# Autodesk Inventor assembly: Model-3
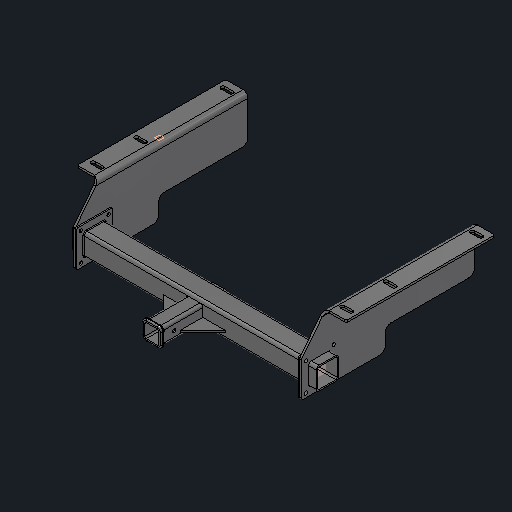
[picture p0: Inventor's stored thumbnail of the model, 512x512]
Saved by Autodesk Inventor 2025.1 (Build 291241000, 241)
## iProperties
Created: 2026-02-13
Part Number: Model-3
Document SubType Name: Assembly
Designer: Desktop -24
Mass: 20583.6 g
Surface Area: 8150.6 cm^2
Volume: 2573.11 cm^3
Density: 7.99949 g/cm^3
encoded128: ÌStandard (in)rÎ
Family: ASSEMBLY
Author: Desktop -24
## Documents named in this file (6)
- F:\OneDrive - nLeague Technologies Private Limited\Desktop\Sharath Chandra\Rear Hitch\Model-3\Model-3.iam
- F:\OneDrive - nLeague Technologies Private Limited\Desktop\Sharath Chandra\Rear Hitch\Model-3\Model-3_Base Tube-1.ipt
- F:\OneDrive - nLeague Technologies Private Limited\Desktop\Sharath Chandra\Rear Hitch\Model-3\Model-3_Sheet-LH.ipt
- F:\OneDrive - nLeague Technologies Private Limited\Desktop\Sharath Chandra\Rear Hitch\Model-3\Model-3_Sheet-RH.ipt
- F:\OneDrive - nLeague Technologies Private Limited\Desktop\Sharath Chandra\Rear Hitch\Model-3\Model-3_Base Tube-2.ipt
- F:\OneDrive - nLeague Technologies Private Limited\Desktop\Sharath Chandra\Rear Hitch\Model-3\Model-3_Sheet Stifferner.ipt
## Components (6 placed, 5 different names)
1. Model-3_Sheet-LH:1 — Mate:14, Flush:13, Flush:14
2. Model-3_Base Tube-1:1 — Mate:4, Mate:5, Flush:2, Mate:8, Mate:10, Mate:13, Flush:11, Flush:12, Mate:14, Flush:13, Flush:14
3. Model-3_Base Tube-2:1 — Mate:4, Mate:5, Flush:2, Mate:9, Mate:11, Flush:8
4. Model-3_Sheet-RH:1 — Mate:13, Flush:11, Flush:12
5. Model-3_Sheet Stifferner:1 — Mate:8, Mate:9, Flush:7
6. Model-3_Sheet Stifferner:2 — Mate:10, Mate:11, Flush:7, Flush:8
## Relationships (15: Mate 8, Flush 7)
- Mate:4: Model-3_Base Tube-1:1 ↔ Model-3_Base Tube-2:1
- Mate:5: Model-3_Base Tube-1:1 ↔ Model-3_Base Tube-2:1
- Flush:2 (9.525 mm): Model-3_Base Tube-1:1 ↔ Model-3_Base Tube-2:1
- Mate:8: Model-3_Base Tube-1:1 ↔ Model-3_Sheet Stifferner:1
- Mate:9: Model-3_Base Tube-2:1 ↔ Model-3_Sheet Stifferner:1
- Mate:10: Model-3_Base Tube-1:1 ↔ Model-3_Sheet Stifferner:2
- Mate:11: Model-3_Base Tube-2:1 ↔ Model-3_Sheet Stifferner:2
- Flush:7: Model-3_Sheet Stifferner:1 ↔ Model-3_Sheet Stifferner:2
- Flush:8 (-50.8 mm): Model-3_Base Tube-2:1 ↔ Model-3_Sheet Stifferner:2
- Mate:13: Model-3_Base Tube-1:1 ↔ Model-3_Sheet-RH:1
- Flush:11: Model-3_Base Tube-1:1 ↔ Model-3_Sheet-RH:1
- Flush:12: Model-3_Base Tube-1:1 ↔ Model-3_Sheet-RH:1
- Mate:14: Model-3_Sheet-LH:1 ↔ Model-3_Base Tube-1:1
- Flush:13: Model-3_Sheet-LH:1 ↔ Model-3_Base Tube-1:1
- Flush:14: Model-3_Sheet-LH:1 ↔ Model-3_Base Tube-1:1
